# Autodesk Inventor assembly: V-Slot Delrin Dual Wheel Assembly
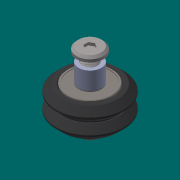
[picture p0: Inventor's stored thumbnail of the model, 180x180]
Saved by Autodesk Inventor 2016 (Build 200138000, 138)
## iProperties
Created: 2015-02-28
Part Number: V-Slot Delrin Dual Wheel Assembly
Document SubType Name: Assembly
Designer: Sawaiz Syed
Author: Mark
Title: V-Slot Delrin Dual Wheel Assembly.step
Description: STEP AP214
Creation Date: 2015-01-21
Sending System: SolidWorks 2013
Preprocessor: SwSTEP 2.0
Author: Sawaiz Syed
## Documents named in this file (7)
- C:\Users\Sawaiz\Documents\data\projects\cncBlackBox\vWheel\V-Slot Delrin Dual Wheel Assembly.iam
- C:\Users\Sawaiz\Documents\data\projects\cncBlackBox\hardware\delrinVWheel.ipt
- C:\Users\Sawaiz\Documents\data\projects\cncBlackBox\hardware\625BallBearing.ipt
- C:\Users\Sawaiz\Documents\data\projects\cncBlackBox\hardware\m5PrecisionWasher.ipt
- C:\Users\Sawaiz\Documents\data\projects\cncBlackBox\hardware\0.25inSpacer.ipt
- C:\Users\Sawaiz\Documents\data\projects\cncBlackBox\hardware\m5x25LowProfile.ipt
- C:\Users\Sawaiz\Documents\data\projects\cncBlackBox\hardware\m5Nylock.ipt
## Components (7 placed, 7 different names)
1. delrinVWheel — Mate:6, Mate:7, Mate:8, Mate:9, Mate:11
2. 625BallBearingTop — Mate:2, Mate:3, Mate:4, Mate:5, Mate:6
3. 625BallBearingBottom — Mate:8, Mate:9, Mate:12
4. m5PrecisionWasher — Mate:3, Mate:4
5. 0.25inSpacer — Mate:1, Mate:2, Mate:5, Mate:7, Mate:10
6. m5x25LowProfile — Mate:1, Mate:10
7. m5Nylock — Mate:11, Mate:12
## Relationships (12: Mate 12)
- Mate:1: 0.25inSpacer ↔ m5x25LowProfile
- Mate:2: 625BallBearingTop ↔ 0.25inSpacer
- Mate:3: 625BallBearingTop ↔ m5PrecisionWasher
- Mate:4: 625BallBearingTop ↔ m5PrecisionWasher
- Mate:5: 625BallBearingTop ↔ 0.25inSpacer
- Mate:6: delrinVWheel ↔ 625BallBearingTop
- Mate:7: delrinVWheel ↔ 0.25inSpacer
- Mate:8: delrinVWheel ↔ 625BallBearingBottom
- Mate:9: delrinVWheel ↔ 625BallBearingBottom
- Mate:10 (3 mm): 0.25inSpacer ↔ m5x25LowProfile
- Mate:11: delrinVWheel ↔ m5Nylock
- Mate:12: 625BallBearingBottom ↔ m5Nylock
